# Autodesk Inventor assembly: Full PC104 ISA Low Profile2
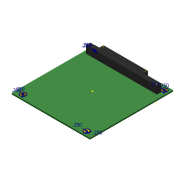
[picture p0: Inventor's stored thumbnail of the model, 180x180]
Saved by Autodesk Inventor 2018 (Build 220112000, 112)
## iProperties
Created: 2018-12-12
Part Number: Full PC104 ISA Low Profile2
Document SubType Name: Assembly
Designer: R.P.SMITH
Mass: 21.71 g
Surface Area: 250.171 cm^2
Volume: 19.1442 cm^3
Density: 1.13403 g/cm^3
Author: R.P.SMITH
## Documents named in this file (4)
- D:\Documents\College\Semesters\4 - Fall\Senior Project 2\CADD Files\PC104 ISA BOARD ULTRA LOW PROFILE.iam
- D:\Documents\College\Semesters\4 - Fall\Senior Project 2\CADD Files\Custom Parts\PC104 ISA BUS.ipt
- D:\Documents\College\Semesters\4 - Fall\Senior Project 2\CADD Files\Mouser\SSQ-132-22-G-D.ipt
- D:\Documents\College\Semesters\4 - Fall\Senior Project 2\CADD Files\Mouser\SSQ-120-22-G-D.ipt
## Components (3 placed, 3 different names)
1. PC104 ISA BUS:1 — Mate:1, Mate:2, Mate:3, Mate:4, Mate:5, Mate:6
2. SSQ-132-22-G-D:1 — Mate:1, Mate:2, Mate:3
3. SSQ-120-22-G-D:1 — Mate:4, Mate:5, Mate:6
## Relationships (6: Mate 6)
- Mate:1: PC104 ISA BUS:1 ↔ SSQ-132-22-G-D:1
- Mate:2: PC104 ISA BUS:1 ↔ SSQ-132-22-G-D:1
- Mate:3: PC104 ISA BUS:1 ↔ SSQ-132-22-G-D:1
- Mate:4: PC104 ISA BUS:1 ↔ SSQ-120-22-G-D:1
- Mate:5: PC104 ISA BUS:1 ↔ SSQ-120-22-G-D:1
- Mate:6: PC104 ISA BUS:1 ↔ SSQ-120-22-G-D:1
